# Autodesk Inventor assembly: NewClaw
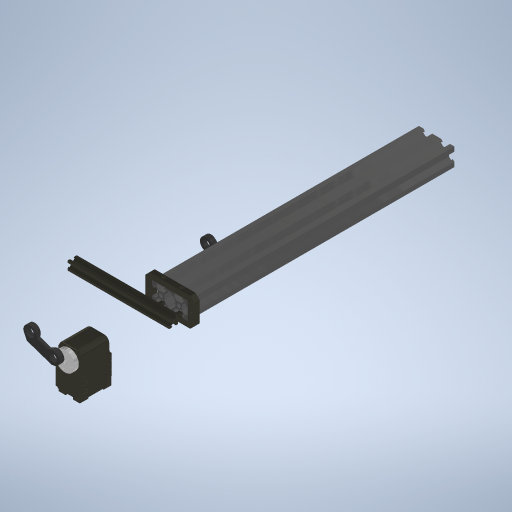
[picture p0: Inventor's stored thumbnail of the model, 512x512]
Saved by Autodesk Inventor 2024.3 (Build 283343000, 343)
## iProperties
Created: 2025-01-07
Part Number: NewClaw
Document SubType Name: Assembly
Designer: migue
Author: migue
## Documents named in this file (9)
- C:\Users\migue\Documents\GitHub\RobotCartesiano\DiseñoMecánico\Assemblies\NewClaw.iam
- C:\Users\migue\Documents\GitHub\RobotCartesiano\DiseñoMecánico\AcrylicPieces\ServoCarrier.ipt
- C:\Users\migue\Documents\GitHub\RobotCartesiano\DiseñoMecánico\Axis\AxisZ\MovingPlate\AP-ZClaw.ipt
- C:\Users\migue\Documents\GitHub\RobotCartesiano\DiseñoMecánico\Axis\AxisZ\MovingPlate\AP10x10.ipt
- C:\Users\migue\Documents\GitHub\RobotCartesiano\DiseñoMecánico\Axis\AxisZ\MovingPlate\MechanismArm.ipt
- C:\Users\migue\Documents\GitHub\RobotCartesiano\DiseñoMecánico\Motors\DynamixelAX12A\Pieces\AX12 middle.STEP.ipt
- C:\Users\migue\Documents\GitHub\RobotCartesiano\DiseñoMecánico\Motors\DynamixelAX12A\Pieces\AX12 Back.STEP.ipt
- C:\Users\migue\Documents\GitHub\RobotCartesiano\DiseñoMecánico\Motors\DynamixelAX12A\Pieces\AX12 Front.STEP.ipt
- C:\Users\migue\Documents\GitHub\RobotCartesiano\DiseñoMecánico\Motors\DynamixelAX12A\Pieces\Axel.STEP.ipt
## Components (9 placed, 8 different names)
1. ServoCarrier:1 — Mate:1, Flush:1, Mate:2
2. AP-ZClaw:1 — Mate:1, Flush:1, Mate:2
3. AP10x10:1
4. MechanismArm:1 — Mate:7, Mate:8
5. MechanismArm:2
6. Axel.STEP:1 — Mate:5, Mate:6, Mate:7, Mate:8
7. AX12 middle.STEP:1 — Mate:3, Flush:2, Flush:3, Flush:4, Mate:4, Flush:5
8. AX12 Back.STEP:1 — Mate:3, Flush:2, Flush:3
9. AX12 Front.STEP:1 — Flush:4, Mate:4, Flush:5, Mate:5, Mate:6
## Relationships (13: Mate 8, Flush 5)
- Mate:1: ServoCarrier:1 ↔ AP-ZClaw:1
- Flush:1: ServoCarrier:1 ↔ AP-ZClaw:1
- Mate:2: ServoCarrier:1 ↔ AP-ZClaw:1
- Mate:3: AX12 middle.STEP:1 ↔ AX12 Back.STEP:1
- Flush:2: AX12 middle.STEP:1 ↔ AX12 Back.STEP:1
- Flush:3: AX12 middle.STEP:1 ↔ AX12 Back.STEP:1
- Flush:4: AX12 middle.STEP:1 ↔ AX12 Front.STEP:1
- Mate:4: AX12 middle.STEP:1 ↔ AX12 Front.STEP:1
- Flush:5: AX12 middle.STEP:1 ↔ AX12 Front.STEP:1
- Mate:5: Axel.STEP:1 ↔ AX12 Front.STEP:1
- Mate:6: Axel.STEP:1 ↔ AX12 Front.STEP:1
- Mate:7: MechanismArm:1 ↔ Axel.STEP:1
- Mate:8: MechanismArm:1 ↔ Axel.STEP:1
